# Autodesk Inventor assembly: Header_With_Dimensions_3.5_x_3.5_x_50.25_Inches
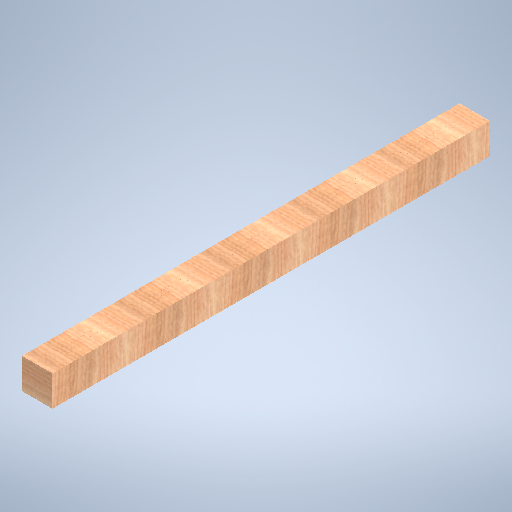
[picture p0: Inventor's stored thumbnail of the model, 512x512]
Saved by Autodesk Inventor 2025 (Build 290162010, 162A)
## iProperties
Created: 2024-10-13
Part Number: Header_With_Dimensions_3.5_x_3.5_x_50.25_Inches
Document SubType Name: Assembly
Designer: Tom
Author: Tom
## Documents named in this file (3)
- C:\Users\Tom\Documents\Inventor\Mobility\Additional_Building\Header_With_Dimensions_3.5_x_3.5_x_50.25_Inches.iam
- C:\Users\Tom\Documents\Inventor\Mobility\Additional_Building\Header_With_Dimensions_1.5_x_3.5_x_50.25_Inches.ipt
- C:\Users\Tom\Documents\Inventor\Mobility\Additional_Building\Header_With_Dimensions_0.5_x_3.5_x_50.25_Inches.ipt
## Components (3 placed, 2 different names)
1. Header_With_Dimensions_1.5_x_3.5_x_50.25_Inches:1 — Mate:1, Flush:1, Flush:2
2. Header_With_Dimensions_1.5_x_3.5_x_50.25_Inches:2 — Mate:2, Flush:3, Flush:4
3. Header_With_Dimensions_0.5_x_3.5_x_50.25_Inches:1 — Mate:1, Flush:1, Flush:2, Mate:2, Flush:3, Flush:4
## Relationships (6: Flush 4, Mate 2)
- Mate:1: Header_With_Dimensions_1.5_x_3.5_x_50.25_Inches:1 ↔ Header_With_Dimensions_0.5_x_3.5_x_50.25_Inches:1
- Flush:1: Header_With_Dimensions_1.5_x_3.5_x_50.25_Inches:1 ↔ Header_With_Dimensions_0.5_x_3.5_x_50.25_Inches:1
- Flush:2: Header_With_Dimensions_1.5_x_3.5_x_50.25_Inches:1 ↔ Header_With_Dimensions_0.5_x_3.5_x_50.25_Inches:1
- Mate:2: Header_With_Dimensions_1.5_x_3.5_x_50.25_Inches:2 ↔ Header_With_Dimensions_0.5_x_3.5_x_50.25_Inches:1
- Flush:3: Header_With_Dimensions_1.5_x_3.5_x_50.25_Inches:2 ↔ Header_With_Dimensions_0.5_x_3.5_x_50.25_Inches:1
- Flush:4: Header_With_Dimensions_1.5_x_3.5_x_50.25_Inches:2 ↔ Header_With_Dimensions_0.5_x_3.5_x_50.25_Inches:1
